# Autodesk Inventor assembly: Rack
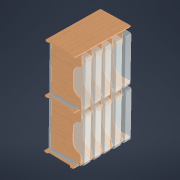
[picture p0: Inventor's stored thumbnail of the model, 180x180]
Saved by Autodesk Inventor 2021 (Build 250183000, 183)
## iProperties
Created: 2023-03-30
Part Number: Rack
Document SubType Name: Assembly
Designer: casey
Author: casey
## Documents named in this file (6)
- E:\casey\dev\Rack\Rack.iam
- E:\casey\dev\Rack\parts\box.ipt
- E:\casey\dev\Rack\parts\slide_panel.ipt
- E:\casey\dev\Rack\parts\slide_panel_back_stopper.ipt
- E:\casey\dev\Rack\parts\slide_panel_joint.ipt
- E:\casey\dev\Rack\parts\side_panel.ipt
## Components (53 placed, 5 different names)
1. box:1
2. slide_panel:1 — 挿入:1, 挿入:2, 挿入:3, 挿入:4, 挿入:5, 挿入:6, 挿入:7, 挿入:8
3. slide_panel_back_stopper:1 — 挿入:1, 挿入:4, 挿入:8
4. slide_panel_joint:1 — 挿入:2, 挿入:3, 挿入:7
5. slide_panel_joint:2 — 挿入:5, 挿入:6, 挿入:9, 挿入:10
6. side_panel:1 — 挿入:9, 挿入:10, 挿入:19, 挿入:20, 挿入:37, 挿入:38, 挿入:39, 挿入:40, 挿入:49, 挿入:50
7. slide_panel:2
8. slide_panel_back_stopper:2
9. slide_panel_joint:3
10. slide_panel_joint:4 — 挿入:19, 挿入:20
11. slide_panel:3
12. slide_panel_back_stopper:3
13. slide_panel_joint:5
14. slide_panel_joint:6 — 挿入:37, 挿入:38
15. slide_panel:4
16. slide_panel_back_stopper:4
17. slide_panel_joint:7
18. slide_panel_joint:8 — 挿入:39, 挿入:40
19. slide_panel:5
20. slide_panel_back_stopper:5
21. slide_panel_joint:9 — 挿入:101, 挿入:102
22. slide_panel_joint:10 — 挿入:49, 挿入:50
23. side_panel:2 — 挿入:103, 挿入:104
24. slide_panel:6
25. slide_panel_back_stopper:6
26. slide_panel_joint:11
27. slide_panel_joint:12
28. side_panel:3 — 挿入:101, 挿入:102
29. slide_panel:7
30. slide_panel_back_stopper:7
31. slide_panel_joint:13
32. slide_panel_joint:14
33. slide_panel:8
34. slide_panel_back_stopper:8
35. slide_panel_joint:15
36. slide_panel_joint:16
37. slide_panel:9
38. slide_panel_back_stopper:9
39. slide_panel_joint:17
40. slide_panel_joint:18
41. slide_panel:10
42. slide_panel_back_stopper:10
43. slide_panel_joint:19 — 挿入:103, 挿入:104
44. slide_panel_joint:20
45. box:2
46. box:3
47. box:4
48. box:5
49. box:6
50. box:7
51. box:8
52. box:9
53. box:10
## Relationships (104: Insert 104)
- 挿入:1 [Insert]: slide_panel:1 ↔ slide_panel_back_stopper:1
- 挿入:2 [Insert]: slide_panel:1 ↔ slide_panel_joint:1
- 挿入:3 [Insert]: slide_panel:1 ↔ slide_panel_joint:1
- 挿入:4 [Insert]: slide_panel:1 ↔ slide_panel_back_stopper:1
- 挿入:5 [Insert]: slide_panel:1 ↔ slide_panel_joint:2
- 挿入:6 [Insert]: slide_panel:1 ↔ slide_panel_joint:2
- 挿入:7 [Insert]: slide_panel:1 ↔ slide_panel_joint:1
- 挿入:8 [Insert]: slide_panel:1 ↔ slide_panel_back_stopper:1
- 挿入:9 [Insert]: slide_panel_joint:2 ↔ side_panel:1
- 挿入:10 [Insert]: slide_panel_joint:2 ↔ side_panel:1
- [Insert]: slide_panel:2 ↔ slide_panel_back_stopper:2
- [Insert]: slide_panel:2 ↔ slide_panel_joint:3
- [Insert]: slide_panel:2 ↔ slide_panel_joint:3
- [Insert]: slide_panel:2 ↔ slide_panel_back_stopper:2
- [Insert]: slide_panel:2 ↔ slide_panel_joint:4
- [Insert]: slide_panel:2 ↔ slide_panel_joint:4
- [Insert]: slide_panel:2 ↔ slide_panel_joint:3
- [Insert]: slide_panel:2 ↔ slide_panel_back_stopper:2
- 挿入:19 [Insert]: side_panel:1 ↔ slide_panel_joint:4
- 挿入:20 [Insert]: side_panel:1 ↔ slide_panel_joint:4
- [Insert]: slide_panel:3 ↔ slide_panel_back_stopper:3
- [Insert]: slide_panel:3 ↔ slide_panel_joint:5
- [Insert]: slide_panel:3 ↔ slide_panel_joint:5
- [Insert]: slide_panel:3 ↔ slide_panel_back_stopper:3
- [Insert]: slide_panel:3 ↔ slide_panel_joint:6
- [Insert]: slide_panel:3 ↔ slide_panel_joint:6
- [Insert]: slide_panel:3 ↔ slide_panel_joint:5
- [Insert]: slide_panel:3 ↔ slide_panel_back_stopper:3
- [Insert]: slide_panel:4 ↔ slide_panel_back_stopper:4
- [Insert]: slide_panel:4 ↔ slide_panel_joint:7
- [Insert]: slide_panel:4 ↔ slide_panel_joint:7
- [Insert]: slide_panel:4 ↔ slide_panel_back_stopper:4
- [Insert]: slide_panel:4 ↔ slide_panel_joint:8
- [Insert]: slide_panel:4 ↔ slide_panel_joint:8
- [Insert]: slide_panel:4 ↔ slide_panel_joint:7
- [Insert]: slide_panel:4 ↔ slide_panel_back_stopper:4
- 挿入:37 [Insert]: side_panel:1 ↔ slide_panel_joint:6
- 挿入:38 [Insert]: side_panel:1 ↔ slide_panel_joint:6
- 挿入:39 [Insert]: side_panel:1 ↔ slide_panel_joint:8
- 挿入:40 [Insert]: side_panel:1 ↔ slide_panel_joint:8
- [Insert]: slide_panel:5 ↔ slide_panel_back_stopper:5
- [Insert]: slide_panel:5 ↔ slide_panel_joint:9
- [Insert]: slide_panel:5 ↔ slide_panel_joint:9
- [Insert]: slide_panel:5 ↔ slide_panel_back_stopper:5
- [Insert]: slide_panel:5 ↔ slide_panel_joint:10
- [Insert]: slide_panel:5 ↔ slide_panel_joint:10
- [Insert]: slide_panel:5 ↔ slide_panel_joint:9
- [Insert]: slide_panel:5 ↔ slide_panel_back_stopper:5
- 挿入:49 [Insert]: side_panel:1 ↔ slide_panel_joint:10
- 挿入:50 [Insert]: side_panel:1 ↔ slide_panel_joint:10
- [Insert]: slide_panel:6 ↔ slide_panel_back_stopper:6
- [Insert]: slide_panel:6 ↔ slide_panel_joint:11
- [Insert]: slide_panel:6 ↔ slide_panel_joint:11
- [Insert]: slide_panel:6 ↔ slide_panel_back_stopper:6
- [Insert]: slide_panel:6 ↔ slide_panel_joint:12
- [Insert]: slide_panel:6 ↔ slide_panel_joint:12
- [Insert]: slide_panel:6 ↔ slide_panel_joint:11
- [Insert]: slide_panel:6 ↔ slide_panel_back_stopper:6
- [Insert]: slide_panel_joint:12 ↔ side_panel:3
- [Insert]: slide_panel_joint:12 ↔ side_panel:3
- [Insert]: slide_panel:7 ↔ slide_panel_back_stopper:7
- [Insert]: slide_panel:7 ↔ slide_panel_joint:13
- [Insert]: slide_panel:7 ↔ slide_panel_joint:13
- [Insert]: slide_panel:7 ↔ slide_panel_back_stopper:7
- [Insert]: slide_panel:7 ↔ slide_panel_joint:14
- [Insert]: slide_panel:7 ↔ slide_panel_joint:14
- [Insert]: slide_panel:7 ↔ slide_panel_joint:13
- [Insert]: slide_panel:7 ↔ slide_panel_back_stopper:7
- [Insert]: side_panel:3 ↔ slide_panel_joint:14
- [Insert]: side_panel:3 ↔ slide_panel_joint:14
- [Insert]: slide_panel:8 ↔ slide_panel_back_stopper:8
- [Insert]: slide_panel:8 ↔ slide_panel_joint:15
- [Insert]: slide_panel:8 ↔ slide_panel_joint:15
- [Insert]: slide_panel:8 ↔ slide_panel_back_stopper:8
- [Insert]: slide_panel:8 ↔ slide_panel_joint:16
- [Insert]: slide_panel:8 ↔ slide_panel_joint:16
- [Insert]: slide_panel:8 ↔ slide_panel_joint:15
- [Insert]: slide_panel:8 ↔ slide_panel_back_stopper:8
- [Insert]: slide_panel:9 ↔ slide_panel_back_stopper:9
- [Insert]: slide_panel:9 ↔ slide_panel_joint:17
- [Insert]: slide_panel:9 ↔ slide_panel_joint:17
- [Insert]: slide_panel:9 ↔ slide_panel_back_stopper:9
- [Insert]: slide_panel:9 ↔ slide_panel_joint:18
- [Insert]: slide_panel:9 ↔ slide_panel_joint:18
- [Insert]: slide_panel:9 ↔ slide_panel_joint:17
- [Insert]: slide_panel:9 ↔ slide_panel_back_stopper:9
- [Insert]: side_panel:3 ↔ slide_panel_joint:16
- [Insert]: side_panel:3 ↔ slide_panel_joint:16
- [Insert]: side_panel:3 ↔ slide_panel_joint:18
- [Insert]: side_panel:3 ↔ slide_panel_joint:18
- [Insert]: slide_panel:10 ↔ slide_panel_back_stopper:10
- [Insert]: slide_panel:10 ↔ slide_panel_joint:19
- [Insert]: slide_panel:10 ↔ slide_panel_joint:19
- [Insert]: slide_panel:10 ↔ slide_panel_back_stopper:10
- [Insert]: slide_panel:10 ↔ slide_panel_joint:20
- [Insert]: slide_panel:10 ↔ slide_panel_joint:20
- [Insert]: slide_panel:10 ↔ slide_panel_joint:19
- [Insert]: slide_panel:10 ↔ slide_panel_back_stopper:10
- [Insert]: side_panel:3 ↔ slide_panel_joint:20
- [Insert]: side_panel:3 ↔ slide_panel_joint:20
- 挿入:101 [Insert]: slide_panel_joint:9 ↔ side_panel:3
- 挿入:102 [Insert]: slide_panel_joint:9 ↔ side_panel:3
- 挿入:103 [Insert]: side_panel:2 ↔ slide_panel_joint:19
- 挿入:104 [Insert]: side_panel:2 ↔ slide_panel_joint:19
## Named parameters: d14_d6 = 0 mm, d15_d7 = 0 mm, d16_d8 = 0 mm, d17_d9 = 0 mm, d18_d10 = 0 mm, d19_d2 = 0 mm, d20_d4 = 0 mm, d21_d5 = 0 mm, d25_d14_d6 = 0 mm, d26_d15_d7 = 0 mm, d27_d16_d8 = 0 mm, d28_d17_d9 = 0 mm, d29_d18_d10 = 0 mm, d30_d19_d2 = 0 mm, d31_d20_d4 = 0 mm, d32_d21_d5 = 0 mm, d33_d14_d6 = 0 mm, d34_d15_d7 = 0 mm, d35_d16_d8 = 0 mm, d36_d17_d9 = 0 mm, d37_d18_d10 = 0 mm, d38_d19_d2 = 0 mm, d39_d20_d4 = 0 mm, d40_d21_d5 = 0 mm, d45_d14_d6 = 0 mm, d46_d15_d7 = 0 mm, d47_d16_d8 = 0 mm, d48_d17_d9 = 0 mm, d49_d18_d10 = 0 mm, d50_d19_d2 = 0 mm, d51_d20_d4 = 0 mm, d52_d21_d5 = 0 mm, d55_d33_d14_d6 = 0 mm, d56_d34_d15_d7 = 0 mm, d57_d35_d16_d8 = 0 mm, d58_d36_d17_d9 = 0 mm, d59_d37_d18_d10 = 0 mm, d60_d38_d19_d2 = 0 mm, d61_d39_d20_d4 = 0 mm, d62_d40_d21_d5 = 0 mm, d63_d41 = 0 mm, d64_d42 = 0 mm, d65_d43 = 0 mm, d66_d44 = 0 mm, d67_d45_d14_d6 = 0 mm, d68_d46_d15_d7 = 0 mm, d69_d47_d16_d8 = 0 mm, d70_d48_d17_d9 = 0 mm, d71_d49_d18_d10 = 0 mm, d72_d50_d19_d2 = 0 mm, d73_d51_d20_d4 = 0 mm, d74_d52_d21_d5 = 0 mm, d75_d53 = 0 mm, d76_d54 = 0 mm, d77_d6 = 0 mm, d78_d7 = 0 mm, d79_d8 = 0 mm, d80_d9 = 0 mm, d81_d10 = 0 mm, d82_d12 = 0 mm, d83_d13 = 0 mm, d84_d14_d6 = 0 mm, d85_d15_d7 = 0 mm, d86_d16_d8 = 0 mm, d87_d17_d9 = 0 mm, d88_d18_d10 = 0 mm, d89_d19_d2 = 0 mm, d90_d20_d4 = 0 mm, d91_d21_d5 = 0 mm, d92_d23 = 0 mm, d93_d24 = 0 mm, d94_d25_d14_d6 = 0 mm, d95_d26_d15_d7 = 0 mm, d96_d27_d16_d8 = 0 mm, d97_d28_d17_d9 = 0 mm, d98_d29_d18_d10 = 0 mm, d99_d30_d19_d2 = 0 mm, d100_d31_d20_d4 = 0 mm, d101_d32_d21_d5 = 0 mm, d102_d2 = 0 mm, d103_d4 = 0 mm, d104_d5 = 0 mm
